# Autodesk Inventor assembly: Right Wheel
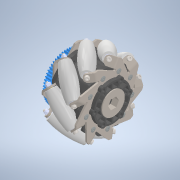
[picture p0: Inventor's stored thumbnail of the model, 180x180]
Saved by Autodesk Inventor 2020 (Build 240168000, 168)
## iProperties
Created: 2022-10-15
Part Number: Right Wheel
Document SubType Name: Assembly
Designer: Jason
Author: Jason
## Documents named in this file (4)
- C:\Users\Jason\Documents\Inventor\FTC Robot 2023\Right Wheel - Back.iam
- C:\Users\Jason\Documents\Inventor\FTC Robot 2023\Wheel Bearing.ipt
- C:\Users\Jason\Documents\Inventor\FTC Robot 2023\FTC Wheel Gear.ipt
- C:\Users\Jason\Documents\Inventor\FTC Robot 2023\Left Wheel.ipt
## Components (4 placed, 3 different names)
1. Left Wheel:1 — Mate:1, Mate:2, Mate:3, Mate:4, Mate:5, Mate:6, Mate:7
2. Spur Gear2:1 — Mate:5, Mate:6, Mate:7
3. Wheel Bearing:1 — Mate:1, Mate:2
4. Wheel Bearing:2 — Mate:3, Mate:4
## Relationships (7: Mate 7)
- Mate:1: Left Wheel:1 ↔ Wheel Bearing:1
- Mate:2: Left Wheel:1 ↔ Wheel Bearing:1
- Mate:3: Left Wheel:1 ↔ Wheel Bearing:2
- Mate:4: Left Wheel:1 ↔ Wheel Bearing:2
- Mate:5: Left Wheel:1 ↔ Spur Gear2:1
- Mate:6: Left Wheel:1 ↔ Spur Gear2:1
- Mate:7: Left Wheel:1 ↔ Spur Gear2:1
